# Autodesk Inventor assembly: RowanSkateBoard
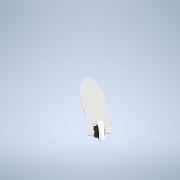
[picture p0: Inventor's stored thumbnail of the model, 180x180]
Saved by Autodesk Inventor 2021 (Build 250183000, 183)
## iProperties
Created: 2021-03-14
Part Number: RowanSkateBoard
Document SubType Name: Assembly
Designer: bl17
Author: bl17
## Documents named in this file (4)
- P:\Personal Docs\RowanSkateBoard\RowanSkateBoard.iam
- P:\Personal Docs\RowanSkateBoard\Board.ipt
- P:\Personal Docs\RowanSkateBoard\Downloaded Parts\SlottedAngles\1.5 Slotted Angle Bar.ipt
- P:\Personal Docs\RowanSkateBoard\Downloaded Parts\002. DC Brushed Wheels.ipt
## Components (4 placed, 3 different names)
1. Board:1 — Flush:1, Mate:1, Mate:2, Mate:3
2. 1.5 Slotted Angle Bar:1 — Flush:1, Mate:1, Mate:2, Mate:4, Mate:5, Mate:6, Mate:7
3. 1.5 Slotted Angle Bar:2 — Mate:3, Mate:4, Mate:5
4. 002. DC Brushed Wheels:1 — Mate:6, Mate:7
## Relationships (8: Mate 7, Flush 1)
- Flush:1: Board:1 ↔ 1.5 Slotted Angle Bar:1
- Mate:1: Board:1 ↔ 1.5 Slotted Angle Bar:1
- Mate:2: Board:1 ↔ 1.5 Slotted Angle Bar:1
- Mate:3: Board:1 ↔ 1.5 Slotted Angle Bar:2
- Mate:4: 1.5 Slotted Angle Bar:1 ↔ 1.5 Slotted Angle Bar:2
- Mate:5 (133.35 mm): 1.5 Slotted Angle Bar:1 ↔ 1.5 Slotted Angle Bar:2
- Mate:6: 1.5 Slotted Angle Bar:1 ↔ 002. DC Brushed Wheels:1
- Mate:7 (14.2875 mm): 1.5 Slotted Angle Bar:1 ↔ 002. DC Brushed Wheels:1
